# Autodesk Inventor assembly: Drone V1
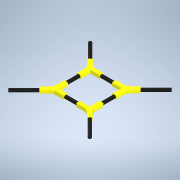
[picture p0: Inventor's stored thumbnail of the model, 180x180]
Saved by Autodesk Inventor 2022 (Build 260153000, 153)
## iProperties
Created: 2022-02-02
Part Number: Drone V1
Document SubType Name: Assembly
Designer: ultra
Author: ultra
## Documents named in this file (3)
- C:\Users\ultra\Desktop\RAS Aerial\Drone V1.iam
- C:\Users\ultra\Desktop\RAS Aerial\Tube.ipt
- C:\Users\ultra\Desktop\RAS Aerial\BracketV1.ipt
## Components (12 placed, 2 different names)
1. Tube:1 — Insert:1
2. BracketV1:1 — Insert:1, Insert:2, Insert:13
3. Tube:2 — Insert:2, Insert:3
4. BracketV1:3 — Insert:3, Insert:6, Insert:12
5. Tube:4 — Insert:6, Insert:9
6. BracketV1:5 — Insert:9, Flush:1, Insert:11
7. Tube:5
8. BracketV1:6 — Flush:1, Insert:10
9. Tube:6 — Insert:10
10. Tube:7 — Insert:11
11. Tube:8 — Insert:12
12. Tube:9 — Insert:13
## Relationships (12: Insert 11, Flush 1)
- Insert:1: Tube:1 ↔ BracketV1:1
- Insert:2: BracketV1:1 ↔ Tube:2
- Insert:3: Tube:2 ↔ BracketV1:3
- Insert:6: BracketV1:3 ↔ Tube:4
- [Insert]: BracketV1:5 ↔ Tube:5
- [Insert]: Tube:5 ↔ BracketV1:6
- Insert:9: Tube:4 ↔ BracketV1:5
- Flush:1: BracketV1:5 ↔ BracketV1:6
- Insert:10: BracketV1:6 ↔ Tube:6
- Insert:11: BracketV1:5 ↔ Tube:7
- Insert:12: BracketV1:3 ↔ Tube:8
- Insert:13: BracketV1:1 ↔ Tube:9
## Named parameters: d8_d1 = 0 mm, d9_d4 = 0 mm
